# Autodesk Inventor assembly: Bot 1
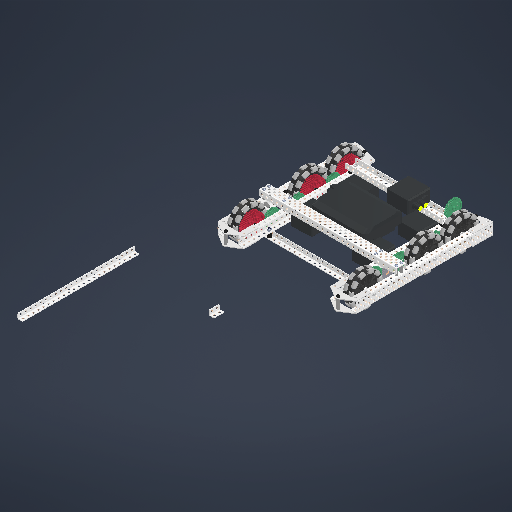
[picture p0: Inventor's stored thumbnail of the model, 512x512]
Saved by Autodesk Inventor 2025.2 (Build 292293000, 293)
## iProperties
Created: 2025-03-17
Part Number: Bot 1
Document SubType Name: Assembly
Designer: Jahan
Author: Jahan
## Documents named in this file (39)
- C:\1629X-7700R-Worlds-Bot\Bot 1\Bot 1.iam
- C:\1629X-7700R-Worlds-Bot\VEX-CAD-Inventor-1.4.2\Structure\C Channel\Aluminum 1x2x1\Alu C 1x2x1x27.ipt
- C:\1629X-7700R-Worlds-Bot\VEX-CAD-Inventor-1.4.2\Structure\C Channel\Aluminum 1x2x1\Alu C 1x2x1x19.ipt
- C:\1629X-7700R-Worlds-Bot\VEX-CAD-Inventor-1.4.2\Motion\Gears\HS Gear.iam
- C:\1629X-7700R-Worlds-Bot\VEX-CAD-Inventor-1.4.2\Motion\Wheels\Omni Wheel\3.25 Omni AS, No Insert.iam
- C:\1629X-7700R-Worlds-Bot\VEX-CAD-Inventor-1.4.2\Motion\Wheels\Omni Wheel.iam
- C:\1629X-7700R-Worlds-Bot\VEX-CAD-Inventor-1.4.2\Motion\Gears\HS Gear\HS 48T Gear, Circle.iam
- C:\1629X-7700R-Worlds-Bot\VEX-CAD-Inventor-1.4.2\Structure\Standoff.ipt
- C:\1629X-7700R-Worlds-Bot\VEX-CAD-Inventor-1.4.2\Structure\Standoff\Standoff .50.ipt
- C:\1629X-7700R-Worlds-Bot\VEX-CAD-Inventor-1.4.2\Motion\Spacers\Washer Teflon.ipt
- C:\1629X-7700R-Worlds-Bot\VEX-CAD-Inventor-1.4.2\Motion\Spacers\Spacer Nylon .375 OD\NSpacer .375 OD x .125.ipt
- C:\1629X-7700R-Worlds-Bot\VEX-CAD-Inventor-1.4.2\Motion\Spacers\Spacer Nylon .375 OD.ipt
- C:\1629X-7700R-Worlds-Bot\VEX-CAD-Inventor-1.4.2\Motion\Spacers\Washer Teflon\TWasher .375 OD x .06250.ipt
- C:\1629X-7700R-Worlds-Bot\VEX-CAD-Inventor-1.4.2\Structure\Hardware\alu_nylock.ipt
- C:\1629X-7700R-Worlds-Bot\VEX-CAD-Inventor-1.4.2\Motion\Gears\LS 36T Gear.ipt
- C:\1629X-7700R-Worlds-Bot\VEX-CAD-Inventor-1.4.2\Motion\Gears\HS Gear\24T HS Gear Cut.iam
- C:\1629X-7700R-Worlds-Bot\VEX-CAD-Inventor-1.4.2\Motion\Shaft LS\Bearing Flat Low Profile.ipt
- C:\1629X-7700R-Worlds-Bot\VEX-CAD-Inventor-1.4.2\Structure\Hardware\Screw Steel - Hex.ipt
- C:\1629X-7700R-Worlds-Bot\VEX-CAD-Inventor-1.4.2\Structure\Hardware\Screw Steel - Hex\SScrew Hex Smooth 1.750.ipt
- C:\1629X-7700R-Worlds-Bot\VEX-CAD-Inventor-1.4.2\Structure\C Channel\Aluminum 1x2x1\Alu C 1x2x1x26.ipt
- C:\1629X-7700R-Worlds-Bot\VEX-CAD-Inventor-1.4.2\Structure\Hardware\Screw Aluminum - Flat Head\AScrew Flat Head Threaded .250.ipt
- C:\1629X-7700R-Worlds-Bot\VEX-CAD-Inventor-1.4.2\Motion\Spacers\Spacer Nylon .375 OD\NSpacer .375 OD x .250.ipt
- C:\1629X-7700R-Worlds-Bot\VEX-CAD-Inventor-1.4.2\Structure\Standoff\Standoff .75.ipt
- C:\1629X-7700R-Worlds-Bot\VEX-CAD-Inventor-1.4.2\Structure\Hardware\Screw Aluminum - Flat Head\AScrew Flat Head Threaded .500.ipt
- C:\1629X-7700R-Worlds-Bot\VEX-CAD-Inventor-1.4.2\Structure\Hardware\Nut Thin Nylock.ipt
- C:\1629X-7700R-Worlds-Bot\VEX-CAD-Inventor-1.4.2\Structure\Hardware\Screw Steel - Star\SScrew Star Smooth .250.ipt
- C:\1629X-7700R-Worlds-Bot\VEX-CAD-Inventor-1.4.2\Structure\Hardware\Screw Steel - Star.ipt
- C:\1629X-7700R-Worlds-Bot\Bot 1\Plastic\backFunnel.ipt
- C:\1629X-7700R-Worlds-Bot\VEX-CAD-Inventor-1.4.2\Structure\Standoff\Standoff 1.00.ipt
- C:\1629X-7700R-Worlds-Bot\VEX-CAD-Inventor-1.4.2\Structure\Angle\Aluminum 1x1\Alu Angle 1x1x19.ipt
- C:\1629X-7700R-Worlds-Bot\VEX-CAD-Inventor-1.4.2\Motion\Spacers\Spacer Nylon .375 OD\NSpacer .375 OD x .500.ipt
- C:\1629X-7700R-Worlds-Bot\VEX-CAD-Inventor-1.4.2\Structure\Hardware\Screw Steel - Star\SScrew Star Smooth .500.ipt
- C:\1629X-7700R-Worlds-Bot\VEX-CAD-Inventor-1.4.2\Electronics\V5 Simple Motor.ipt
- C:\1629X-7700R-Worlds-Bot\VEX-CAD-Inventor-1.4.2\Structure\Hardware\Screw Steel - Star\SScrew Star Smooth .750.ipt
- C:\1629X-7700R-Worlds-Bot\VEX-CAD-Inventor-1.4.2\Structure\Hardware\Screw Nylon - Flat Head\NScrew Flat Head Threaded .250.ipt
- C:\1629X-7700R-Worlds-Bot\VEX-CAD-Inventor-1.4.2\Electronics\V5 Simple Brain.ipt
- C:\1629X-7700R-Worlds-Bot\Bot 1\Plastic\frontFunnel.ipt
- C:\1629X-7700R-Worlds-Bot\VEX-CAD-Inventor-1.4.2\Structure\Angle\Aluminum 1x1\Alu Angle 1x1x2.ipt
- C:\1629X-7700R-Worlds-Bot\VEX-CAD-Inventor-1.4.2\Structure\Angle\Aluminum 1x1\Alu Angle 1x1x23.ipt
## Components (148 placed, 31 different names)
1. Alu C 1x2x1x26:2 — Insert:19, Insert:32, Insert:40, Insert:72, Insert:73, Insert:74, Insert:84, Insert:85, Insert:105, Insert:106, Insert:130, Insert:132, Insert:141, Insert:142, Insert:143, Insert:144, Insert:151, Insert:152, Insert:163, Mate:8, Flush:1, Insert:164, Insert:165, Insert:169, Insert:181, Insert:186, Insert:206, Insert:210, Insert:213
2. Alu C 1x2x1x26:1 — Insert:5, Insert:6, Insert:59, Insert:66, Insert:67, Insert:75, Insert:76, Insert:77, Insert:86, Insert:87, Insert:107, Insert:108, Insert:125, Insert:126, Insert:139, Insert:140, Insert:145, Insert:146, Insert:147, Insert:148, Insert:149, Insert:150, Insert:182, Insert:184, Insert:204, Insert:211, Insert:212
3. Alu C 1x2x1x27:3 — Insert:5, Insert:6, Insert:7, Insert:8, Insert:9, Insert:10
4. Alu C 1x2x1x27:4 — Insert:7, Insert:8, Insert:52, Insert:58, Insert:65, Insert:81, Insert:82, Insert:83, Insert:127, Insert:128, Insert:170, Insert:171, Insert:172, Insert:173, Insert:183, Insert:203
5. Alu C 1x2x1x27:5 — Insert:9, Insert:10, Insert:25, Insert:31, Insert:39, Insert:43, Insert:44, Insert:45, Insert:46, Insert:78, Insert:79, Insert:80, Insert:129, Insert:131, Insert:166, Insert:167, Insert:168, Insert:180, Insert:205, Insert:208, Insert:209
6. LS 36T Gear:1 — Insert:19, Rotation:5, Rotation:6
7. HS 48T Gear, Circle:3 [sub-assembly] — Mate:1, Rotation:4, Rotation:5
8. 3.25 Omni AS, No Insert:4 [sub-assembly] — Mate:1
9. NSpacer .375 OD x .125:2
10. TWasher .375 OD x .06250:2 — Insert:23
11. alu_nylock:3 — Insert:23, Insert:24
12. Standoff .50:3 — Insert:24, Insert:25
13. HS 48T Gear, Circle:4 [sub-assembly] — Mate:2, Rotation:6
14. 3.25 Omni AS, No Insert:5 [sub-assembly] — Mate:2
15. NSpacer .375 OD x .125:3
16. TWasher .375 OD x .06250:3
17. alu_nylock:4
18. Standoff .50:4 — Insert:31
19. LS 36T Gear:2 — Insert:32, Rotation:4
20. HS 48T Gear, Circle:5 [sub-assembly] — Mate:3, Rotation:1
21. 3.25 Omni AS, No Insert:6 [sub-assembly] — Mate:3
22. NSpacer .375 OD x .125:4
23. TWasher .375 OD x .06250:4
24. alu_nylock:5
25. Standoff .50:5 — Insert:39
26. LS 36T Gear:4 — Insert:40, Rotation:1
27. Bearing Flat Low Profile:1 — Insert:43, Insert:44
28. Bearing Flat Low Profile:2 — Insert:45, Insert:46
29. HS 48T Gear, Circle:6 [sub-assembly]
30. 3.25 Omni AS, No Insert:7 [sub-assembly]
31. NSpacer .375 OD x .125:6
32. TWasher .375 OD x .06250:5
33. alu_nylock:6
34. Standoff .50:6 — Insert:52
35. HS 48T Gear, Circle:7 [sub-assembly]
36. 3.25 Omni AS, No Insert:8 [sub-assembly]
37. NSpacer .375 OD x .125:7
38. TWasher .375 OD x .06250:6
39. alu_nylock:7
40. Standoff .50:7 — Insert:58
41. LS 36T Gear:5 — Insert:59
42. HS 48T Gear, Circle:8 [sub-assembly]
43. 3.25 Omni AS, No Insert:9 [sub-assembly]
44. NSpacer .375 OD x .125:8
45. TWasher .375 OD x .06250:7
46. alu_nylock:8
47. Standoff .50:8 — Insert:65
48. LS 36T Gear:6 — Insert:66
49. LS 36T Gear:7 — Insert:67
50. SScrew Hex Smooth 1.750:1 — Insert:72
51. SScrew Hex Smooth 1.750:2 — Insert:74
52. SScrew Hex Smooth 1.750:3 — Insert:73
53. SScrew Hex Smooth 1.750:4 — Insert:77
54. SScrew Hex Smooth 1.750:5 — Insert:76
55. SScrew Hex Smooth 1.750:6 — Insert:75
56. AScrew Flat Head Threaded .250:1 — Insert:78
57. AScrew Flat Head Threaded .250:2 — Insert:79
58. AScrew Flat Head Threaded .250:3 — Insert:80
59. AScrew Flat Head Threaded .250:4 — Insert:81
60. AScrew Flat Head Threaded .250:5 — Insert:82
61. AScrew Flat Head Threaded .250:6 — Insert:83
62. Alu C 1x2x1x19:1 — Insert:88, Insert:89, Insert:90, Mate:7, Insert:101, Insert:102, Insert:103, Insert:104
63. NSpacer .375 OD x .250:10 — Insert:84, Insert:88
64. NSpacer .375 OD x .250:11 — Insert:86, Insert:89
65. NSpacer .375 OD x .250:12 — Insert:87, Insert:90
66. NSpacer .375 OD x .250:13 — Insert:85, Mate:7
67. AScrew Flat Head Threaded .500:1 — Insert:101
68. AScrew Flat Head Threaded .500:2 — Insert:104
69. AScrew Flat Head Threaded .500:3 — Insert:102
70. AScrew Flat Head Threaded .500:4 — Insert:103
71. Nut Thin Nylock:1 — Insert:105
72. Nut Thin Nylock:2 — Insert:108
73. Nut Thin Nylock:3 — Insert:106
74. Nut Thin Nylock:4 — Insert:107
75. backFunnel:1 — Insert:125, Insert:127, Insert:159
76. backFunnel:2 — Insert:126, Insert:128, Insert:133, Insert:160
77. backFunnel:3 — Insert:129, Insert:130, Insert:161
78. backFunnel:4 — Insert:131, Insert:132, Insert:134, Insert:162
79. Standoff 1.00:17 — Insert:134
80. Standoff 1.00:18 — Insert:133
81. SScrew Star Smooth .500:17 — Insert:141
82. SScrew Star Smooth .500:18 — Insert:146
83. SScrew Star Smooth .500:19 — Insert:144
84. SScrew Star Smooth .500:20 — Insert:145
85. SScrew Star Smooth .500:21 — Insert:143
86. SScrew Star Smooth .500:22 — Insert:139
87. SScrew Star Smooth .500:23 — Insert:140
88. SScrew Star Smooth .500:24 — Insert:142
89. V5 Simple Motor:1 — Insert:147, Insert:148
90. V5 Simple Motor:2 — Insert:149, Insert:150
91. V5 Simple Motor:4 — Insert:151, Insert:152
92. SScrew Star Smooth .750:26 — Insert:189
93. NScrew Flat Head Threaded .250:1 — Insert:159
94. NScrew Flat Head Threaded .250:2 — Insert:160
95. NScrew Flat Head Threaded .250:3 — Insert:162
96. NScrew Flat Head Threaded .250:4 — Insert:161
97. V5 Simple Motor:5 — Insert:163, Mate:8
98. V5 Simple Brain:1
99. frontFunnel:1 — Insert:164, Insert:165, Insert:166, Insert:167, Insert:177
100. frontFunnel:2 — Insert:168, Insert:169, Insert:178, Insert:179
101. frontFunnel:3 — Insert:170, Insert:171, Insert:175
102. frontFunnel:4 — Insert:172, Insert:173, Insert:174, Insert:176
103. Standoff 1.00:19 — Insert:179
104. NScrew Flat Head Threaded .250:5 — Insert:177
105. NScrew Flat Head Threaded .250:6 — Insert:178
106. Standoff 1.00:20 — Insert:176
107. NScrew Flat Head Threaded .250:7 — Insert:174
108. NScrew Flat Head Threaded .250:8 — Insert:175
109. Standoff .75:21 — Mate:13
110. Standoff .75:22 — Mate:16, Insert:209
111. SScrew Star Smooth .250:27 — Mate:14
112. SScrew Star Smooth .250:28 — Mate:15
113. SScrew Star Smooth .250:29 — Mate:12
114. SScrew Star Smooth .250:30 — Mate:11
115. Standoff .75:23 — Mate:10
116. Standoff .75:24 — Mate:9
117. Standoff .75:25 — Insert:197
118. Standoff .75:26 — Insert:196
119. Standoff .75:27 — Insert:193
120. Standoff .75:28 — Insert:192
121. Alu C 1x2x1x27:6 — Insert:192, Insert:193, Insert:194, Insert:195, Insert:196, Insert:197, Insert:198, Insert:199, Mate:9, Mate:10, Mate:11, Mate:12, Mate:13, Mate:14, Mate:15, Mate:16, Insert:207
122. SScrew Star Smooth .250:31 — Insert:198
123. SScrew Star Smooth .250:32 — Insert:199
124. SScrew Star Smooth .250:33 — Insert:195
125. SScrew Star Smooth .250:34 — Insert:194
126. SScrew Star Smooth .250:35 — Insert:181
127. SScrew Star Smooth .250:36 — Insert:180
128. SScrew Star Smooth .250:37 — Insert:182
129. SScrew Star Smooth .250:39 — Insert:183
130. NSpacer .375 OD x .125:16 — Insert:184, Insert:185
131. 24T HS Gear Cut:6 [sub-assembly] — Insert:185
132. 24T HS Gear Cut:7 [sub-assembly] — Insert:187
133. NSpacer .375 OD x .125:17 — Insert:186, Insert:187
134. Nut Thin Nylock:6 — Insert:212
135. NSpacer .375 OD x .500:18 — Insert:190, Insert:211
136. Alu Angle 1x1x19:1 — Insert:188, Insert:189, Insert:190, Insert:191
137. NSpacer .375 OD x .500:19 — Insert:191, Insert:210
138. SScrew Star Smooth .750:40 — Insert:188
139. Alu Angle 1x1x2:1
140. Alu Angle 1x1x23:1
141. V5 Simple Motor:9
142. LS 36T Gear:10
143. SScrew Star Smooth .250:41 — Insert:203
144. SScrew Star Smooth .250:42 — Insert:204
145. Standoff .75:29 — Insert:207, Insert:208
146. SScrew Star Smooth .250:43 — Insert:206
147. SScrew Star Smooth .250:44 — Insert:205
148. Nut Thin Nylock:7 — Insert:213
## Relationships (176: Insert 155, Mate 16, RelateRotation 4, Flush 1)
- Insert:5: Alu C 1x2x1x26:1 ↔ Alu C 1x2x1x27:3
- Insert:6: Alu C 1x2x1x26:1 ↔ Alu C 1x2x1x27:3
- Insert:7: Alu C 1x2x1x27:3 ↔ Alu C 1x2x1x27:4
- Insert:8: Alu C 1x2x1x27:3 ↔ Alu C 1x2x1x27:4
- Insert:9: Alu C 1x2x1x27:3 ↔ Alu C 1x2x1x27:5
- Insert:10: Alu C 1x2x1x27:3 ↔ Alu C 1x2x1x27:5
- Insert:19: Alu C 1x2x1x26:2 ↔ LS 36T Gear:1
- [Insert]: HS 48T Gear, Circle:3 ↔ 3.25 Omni AS, No Insert:4
- [Insert]: HS 48T Gear, Circle:3 ↔ NSpacer .375 OD x .125:2
- [Insert]: 3.25 Omni AS, No Insert:4 ↔ TWasher .375 OD x .06250:2
- Insert:23: TWasher .375 OD x .06250:2 ↔ alu_nylock:3
- Insert:24: alu_nylock:3 ↔ Standoff .50:3
- Insert:25: Alu C 1x2x1x27:5 ↔ Standoff .50:3
- [Insert]: HS 48T Gear, Circle:4 ↔ 3.25 Omni AS, No Insert:5
- [Insert]: HS 48T Gear, Circle:4 ↔ NSpacer .375 OD x .125:3
- [Insert]: 3.25 Omni AS, No Insert:5 ↔ TWasher .375 OD x .06250:3
- [Insert]: TWasher .375 OD x .06250:3 ↔ alu_nylock:4
- [Insert]: alu_nylock:4 ↔ Standoff .50:4
- Insert:31: Alu C 1x2x1x27:5 ↔ Standoff .50:4
- Insert:32: Alu C 1x2x1x26:2 ↔ LS 36T Gear:2
- [Insert]: HS 48T Gear, Circle:5 ↔ 3.25 Omni AS, No Insert:6
- [Insert]: HS 48T Gear, Circle:5 ↔ NSpacer .375 OD x .125:4
- [Insert]: 3.25 Omni AS, No Insert:6 ↔ TWasher .375 OD x .06250:4
- [Insert]: TWasher .375 OD x .06250:4 ↔ alu_nylock:5
- [Insert]: alu_nylock:5 ↔ Standoff .50:5
- Insert:39: Alu C 1x2x1x27:5 ↔ Standoff .50:5
- Insert:40: Alu C 1x2x1x26:2 ↔ LS 36T Gear:4
- Mate:1: HS 48T Gear, Circle:3 ↔ 3.25 Omni AS, No Insert:4
- Mate:2: HS 48T Gear, Circle:4 ↔ 3.25 Omni AS, No Insert:5
- Mate:3: HS 48T Gear, Circle:5 ↔ 3.25 Omni AS, No Insert:6
- Insert:43: Alu C 1x2x1x27:5 ↔ Bearing Flat Low Profile:1
- Insert:44: Alu C 1x2x1x27:5 ↔ Bearing Flat Low Profile:1
- Insert:45: Alu C 1x2x1x27:5 ↔ Bearing Flat Low Profile:2
- Insert:46: Alu C 1x2x1x27:5 ↔ Bearing Flat Low Profile:2
- [Insert]: HS 48T Gear, Circle:6 ↔ 3.25 Omni AS, No Insert:7
- [Insert]: HS 48T Gear, Circle:6 ↔ NSpacer .375 OD x .125:6
- [Insert]: 3.25 Omni AS, No Insert:7 ↔ TWasher .375 OD x .06250:5
- [Insert]: TWasher .375 OD x .06250:5 ↔ alu_nylock:6
- [Insert]: alu_nylock:6 ↔ Standoff .50:6
- [Mate]: HS 48T Gear, Circle:6 ↔ 3.25 Omni AS, No Insert:7
- Insert:52: Alu C 1x2x1x27:4 ↔ Standoff .50:6
- [Insert]: HS 48T Gear, Circle:7 ↔ 3.25 Omni AS, No Insert:8
- [Insert]: HS 48T Gear, Circle:7 ↔ NSpacer .375 OD x .125:7
- [Insert]: 3.25 Omni AS, No Insert:8 ↔ TWasher .375 OD x .06250:6
- [Insert]: TWasher .375 OD x .06250:6 ↔ alu_nylock:7
- [Insert]: alu_nylock:7 ↔ Standoff .50:7
- [Mate]: HS 48T Gear, Circle:7 ↔ 3.25 Omni AS, No Insert:8
- Insert:58: Alu C 1x2x1x27:4 ↔ Standoff .50:7
- Insert:59: Alu C 1x2x1x26:1 ↔ LS 36T Gear:5
- [Insert]: HS 48T Gear, Circle:8 ↔ 3.25 Omni AS, No Insert:9
- [Insert]: HS 48T Gear, Circle:8 ↔ NSpacer .375 OD x .125:8
- [Insert]: 3.25 Omni AS, No Insert:9 ↔ TWasher .375 OD x .06250:7
- [Insert]: TWasher .375 OD x .06250:7 ↔ alu_nylock:8
- [Insert]: alu_nylock:8 ↔ Standoff .50:8
- [Mate]: HS 48T Gear, Circle:8 ↔ 3.25 Omni AS, No Insert:9
- Insert:65: Alu C 1x2x1x27:4 ↔ Standoff .50:8
- Insert:66: Alu C 1x2x1x26:1 ↔ LS 36T Gear:6
- Insert:67: Alu C 1x2x1x26:1 ↔ LS 36T Gear:7
- Insert:72: Alu C 1x2x1x26:2 ↔ SScrew Hex Smooth 1.750:1
- Insert:73: Alu C 1x2x1x26:2 ↔ SScrew Hex Smooth 1.750:3
- Insert:74: Alu C 1x2x1x26:2 ↔ SScrew Hex Smooth 1.750:2
- Insert:75: Alu C 1x2x1x26:1 ↔ SScrew Hex Smooth 1.750:6
- Insert:76: Alu C 1x2x1x26:1 ↔ SScrew Hex Smooth 1.750:5
- Insert:77: Alu C 1x2x1x26:1 ↔ SScrew Hex Smooth 1.750:4
- Insert:78: Alu C 1x2x1x27:5 ↔ AScrew Flat Head Threaded .250:1
- Insert:79: Alu C 1x2x1x27:5 ↔ AScrew Flat Head Threaded .250:2
- Insert:80: Alu C 1x2x1x27:5 ↔ AScrew Flat Head Threaded .250:3
- Insert:81: Alu C 1x2x1x27:4 ↔ AScrew Flat Head Threaded .250:4
- Insert:82: Alu C 1x2x1x27:4 ↔ AScrew Flat Head Threaded .250:5
- Insert:83: Alu C 1x2x1x27:4 ↔ AScrew Flat Head Threaded .250:6
- Insert:84: Alu C 1x2x1x26:2 ↔ NSpacer .375 OD x .250:10
- Insert:85: Alu C 1x2x1x26:2 ↔ NSpacer .375 OD x .250:13
- Insert:86: Alu C 1x2x1x26:1 ↔ NSpacer .375 OD x .250:11
- Insert:87: Alu C 1x2x1x26:1 ↔ NSpacer .375 OD x .250:12
- Insert:88: Alu C 1x2x1x19:1 ↔ NSpacer .375 OD x .250:10
- Insert:89: Alu C 1x2x1x19:1 ↔ NSpacer .375 OD x .250:11
- Insert:90: Alu C 1x2x1x19:1 ↔ NSpacer .375 OD x .250:12
- Mate:7: Alu C 1x2x1x19:1 ↔ NSpacer .375 OD x .250:13
- Insert:101: Alu C 1x2x1x19:1 ↔ AScrew Flat Head Threaded .500:1
- Insert:102: Alu C 1x2x1x19:1 ↔ AScrew Flat Head Threaded .500:3
- Insert:103: Alu C 1x2x1x19:1 ↔ AScrew Flat Head Threaded .500:4
- Insert:104: Alu C 1x2x1x19:1 ↔ AScrew Flat Head Threaded .500:2
- Insert:105: Alu C 1x2x1x26:2 ↔ Nut Thin Nylock:1
- Insert:106: Alu C 1x2x1x26:2 ↔ Nut Thin Nylock:3
- Insert:107: Alu C 1x2x1x26:1 ↔ Nut Thin Nylock:4
- Insert:108: Alu C 1x2x1x26:1 ↔ Nut Thin Nylock:2
- Insert:125: Alu C 1x2x1x26:1 ↔ backFunnel:1
- Insert:126: Alu C 1x2x1x26:1 ↔ backFunnel:2
- Insert:127: Alu C 1x2x1x27:4 ↔ backFunnel:1
- Insert:128: Alu C 1x2x1x27:4 ↔ backFunnel:2
- Insert:129: Alu C 1x2x1x27:5 ↔ backFunnel:3
- Insert:130: Alu C 1x2x1x26:2 ↔ backFunnel:3
- Insert:131: Alu C 1x2x1x27:5 ↔ backFunnel:4
- Insert:132: Alu C 1x2x1x26:2 ↔ backFunnel:4
- Insert:133: backFunnel:2 ↔ Standoff 1.00:18
- Insert:134: backFunnel:4 ↔ Standoff 1.00:17
- Insert:139: Alu C 1x2x1x26:1 ↔ SScrew Star Smooth .500:22
- Insert:140: Alu C 1x2x1x26:1 ↔ SScrew Star Smooth .500:23
- Insert:141: Alu C 1x2x1x26:2 ↔ SScrew Star Smooth .500:17
- Insert:142: Alu C 1x2x1x26:2 ↔ SScrew Star Smooth .500:24
- Insert:143: Alu C 1x2x1x26:2 ↔ SScrew Star Smooth .500:21
- Insert:144: Alu C 1x2x1x26:2 ↔ SScrew Star Smooth .500:19
- Insert:145: Alu C 1x2x1x26:1 ↔ SScrew Star Smooth .500:20
- Insert:146: Alu C 1x2x1x26:1 ↔ SScrew Star Smooth .500:18
- Insert:147: Alu C 1x2x1x26:1 ↔ V5 Simple Motor:1
- Insert:148: Alu C 1x2x1x26:1 ↔ V5 Simple Motor:1
- Insert:149: Alu C 1x2x1x26:1 ↔ V5 Simple Motor:2
- Insert:150: Alu C 1x2x1x26:1 ↔ V5 Simple Motor:2
- Insert:151: Alu C 1x2x1x26:2 ↔ V5 Simple Motor:4
- Insert:152: Alu C 1x2x1x26:2 ↔ V5 Simple Motor:4
- Insert:159: backFunnel:1 ↔ NScrew Flat Head Threaded .250:1
- Insert:160: backFunnel:2 ↔ NScrew Flat Head Threaded .250:2
- Insert:161: backFunnel:3 ↔ NScrew Flat Head Threaded .250:4
- Insert:162: backFunnel:4 ↔ NScrew Flat Head Threaded .250:3
- Insert:163: Alu C 1x2x1x26:2 ↔ V5 Simple Motor:5
- Mate:8: Alu C 1x2x1x26:2 ↔ V5 Simple Motor:5
- Flush:1: Alu C 1x2x1x26:2
- Insert:164: Alu C 1x2x1x26:2 ↔ frontFunnel:1
- Insert:165: Alu C 1x2x1x26:2 ↔ frontFunnel:1
- Insert:166: Alu C 1x2x1x27:5 ↔ frontFunnel:1
- Insert:167: Alu C 1x2x1x27:5 ↔ frontFunnel:1
- Insert:168: Alu C 1x2x1x27:5 ↔ frontFunnel:2
- Insert:169: Alu C 1x2x1x26:2 ↔ frontFunnel:2
- Insert:170: Alu C 1x2x1x27:4 ↔ frontFunnel:3
- Insert:171: Alu C 1x2x1x27:4 ↔ frontFunnel:3
- Insert:172: Alu C 1x2x1x27:4 ↔ frontFunnel:4
- Insert:173: Alu C 1x2x1x27:4 ↔ frontFunnel:4
- Insert:174: frontFunnel:4 ↔ NScrew Flat Head Threaded .250:7
- Insert:175: frontFunnel:3 ↔ NScrew Flat Head Threaded .250:8
- Insert:176: frontFunnel:4 ↔ Standoff 1.00:20
- Insert:177: frontFunnel:1 ↔ NScrew Flat Head Threaded .250:5
- Insert:178: frontFunnel:2 ↔ NScrew Flat Head Threaded .250:6
- Insert:179: frontFunnel:2 ↔ Standoff 1.00:19
- Rotation:1 [RelateRotation] (1.3333 ul): HS 48T Gear, Circle:5 ↔ LS 36T Gear:4
- Rotation:4 [RelateRotation] (0.75 ul): HS 48T Gear, Circle:3 ↔ LS 36T Gear:2
- Rotation:5 [RelateRotation] (1.3333 ul): LS 36T Gear:1 ↔ HS 48T Gear, Circle:3
- Rotation:6 [RelateRotation] (0.75 ul): LS 36T Gear:1 ↔ HS 48T Gear, Circle:4
- Insert:180: Alu C 1x2x1x27:5 ↔ SScrew Star Smooth .250:36
- Insert:181: Alu C 1x2x1x26:2 ↔ SScrew Star Smooth .250:35
- Insert:182: Alu C 1x2x1x26:1 ↔ SScrew Star Smooth .250:37
- Insert:183: Alu C 1x2x1x27:4 ↔ SScrew Star Smooth .250:39
- Insert:184: Alu C 1x2x1x26:1 ↔ NSpacer .375 OD x .125:16
- Insert:185: NSpacer .375 OD x .125:16 ↔ 24T HS Gear Cut:6
- Insert:186: Alu C 1x2x1x26:2 ↔ NSpacer .375 OD x .125:17
- Insert:187: 24T HS Gear Cut:7 ↔ NSpacer .375 OD x .125:17
- Insert:188: Alu Angle 1x1x19:1 ↔ SScrew Star Smooth .750:40
- Insert:189: SScrew Star Smooth .750:26 ↔ Alu Angle 1x1x19:1
- Insert:190: NSpacer .375 OD x .500:18 ↔ Alu Angle 1x1x19:1
- Insert:191: Alu Angle 1x1x19:1 ↔ NSpacer .375 OD x .500:19
- Insert:192: Standoff .75:28 ↔ Alu C 1x2x1x27:6
- Insert:193: Standoff .75:27 ↔ Alu C 1x2x1x27:6
- Insert:194: Alu C 1x2x1x27:6 ↔ SScrew Star Smooth .250:34
- Insert:195: Alu C 1x2x1x27:6 ↔ SScrew Star Smooth .250:33
- Insert:196: Standoff .75:26 ↔ Alu C 1x2x1x27:6
- Insert:197: Standoff .75:25 ↔ Alu C 1x2x1x27:6
- Insert:198: Alu C 1x2x1x27:6 ↔ SScrew Star Smooth .250:31
- Insert:199: Alu C 1x2x1x27:6 ↔ SScrew Star Smooth .250:32
- Mate:9: Standoff .75:24 ↔ Alu C 1x2x1x27:6
- Mate:10: Standoff .75:23 ↔ Alu C 1x2x1x27:6
- Mate:11: SScrew Star Smooth .250:30 ↔ Alu C 1x2x1x27:6
- Mate:12: SScrew Star Smooth .250:29 ↔ Alu C 1x2x1x27:6
- Mate:13: Standoff .75:21 ↔ Alu C 1x2x1x27:6
- Mate:14: SScrew Star Smooth .250:27 ↔ Alu C 1x2x1x27:6
- Mate:15: SScrew Star Smooth .250:28 ↔ Alu C 1x2x1x27:6
- Mate:16: Standoff .75:22 ↔ Alu C 1x2x1x27:6
- Insert:203: Alu C 1x2x1x27:4 ↔ SScrew Star Smooth .250:41
- Insert:204: Alu C 1x2x1x26:1 ↔ SScrew Star Smooth .250:42
- Insert:205: Alu C 1x2x1x27:5 ↔ SScrew Star Smooth .250:44
- Insert:206: Alu C 1x2x1x26:2 ↔ SScrew Star Smooth .250:43
- Insert:207: Alu C 1x2x1x27:6 ↔ Standoff .75:29
- Insert:208: Alu C 1x2x1x27:5 ↔ Standoff .75:29
- Insert:209: Alu C 1x2x1x27:5 ↔ Standoff .75:22
- Insert:210: Alu C 1x2x1x26:2 ↔ NSpacer .375 OD x .500:19
- Insert:211: Alu C 1x2x1x26:1 ↔ NSpacer .375 OD x .500:18
- Insert:212: Alu C 1x2x1x26:1 ↔ Nut Thin Nylock:6
- Insert:213: Alu C 1x2x1x26:2 ↔ Nut Thin Nylock:7
## Named parameters: d122_d116 = 0 mm, d123_d117 = 0 mm, d124_d119 = 0 mm, d129_d122_d116 = 0 mm, d130_d123_d117 = 0 mm, d131_d124_d119 = 0 mm, d132_d126 = 0 mm, d133_d127 = 0 mm, d144_d129_d122_d116 = 0 mm, d145_d130_d123_d117 = 0 mm, d146_d131_d124_d119 = 0 mm, d147_d132_d126 = 0 mm, d148_d133_d127 = 0 mm, d162_d127 = 0 mm, d163_d153 = 0 mm, d164_d122_d116 = 0 mm, d165_d123_d117 = 0 mm, d166_d124_d119 = 0 mm, d167_d126 = 0 mm, d169_d127 = 0 mm, d170_d153 = 0 mm, d171_d122_d116 = 0 mm, d172_d123_d117 = 0 mm, d173_d124_d119 = 0 mm, d174_d126 = 0 mm, d177_d169_d127 = 0 mm, d178_d170_d153 = 0 mm, d179_d171_d122_d116 = 0 mm, d180_d172_d123_d117 = 0 mm, d181_d173_d124_d119 = 0 mm, d182_d174_d126 = 0 mm
